# Autodesk Inventor assembly: Track Design 9-24-19
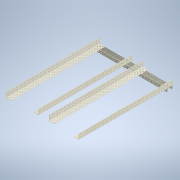
[picture p0: Inventor's stored thumbnail of the model, 180x180]
Saved by Autodesk Inventor 2020 (Build 240168000, 168)
## iProperties
Created: 2019-07-25
Part Number: Track Design 9-24-19
Document SubType Name: Assembly
Designer: Corey
Author: Corey
## Documents named in this file (3)
- C:\Users\Corey\Documents\Tower-Takeover-CAD\Parts\Dual Track.iam
- C:\Users\Corey\Documents\Tower-Takeover-CAD\Parts\Structure\90 Degree Brackets\Aluminum\Aluminum Angle 2x2x35.ipt
- C:\Users\Corey\Documents\Tower-Takeover-CAD\Parts\Structure\C-Channels\Aluminum\2-Wide\Aluminum C-Channel 1x2x1x27.ipt
## Components (5 placed, 2 different names)
1. Aluminum Angle 2x2x35:1 — Mate:6, Flush:11, Flush:12
2. Aluminum Angle 2x2x35:2 — Flush:17, Flush:18
3. Aluminum Angle 2x2x35:3 — Flush:15, Flush:16
4. Aluminum Angle 2x2x35:4
5. Aluminum C-Channel 1x2x1x27:1 — Mate:6, Flush:11, Flush:12, Flush:15, Flush:16, Flush:17, Flush:18
## Relationships (7: Flush 6, Mate 1)
- Mate:6: Aluminum Angle 2x2x35:1 ↔ Aluminum C-Channel 1x2x1x27:1
- Flush:11: Aluminum Angle 2x2x35:1 ↔ Aluminum C-Channel 1x2x1x27:1
- Flush:12: Aluminum Angle 2x2x35:1 ↔ Aluminum C-Channel 1x2x1x27:1
- Flush:15: Aluminum Angle 2x2x35:3 ↔ Aluminum C-Channel 1x2x1x27:1
- Flush:16: Aluminum Angle 2x2x35:3 ↔ Aluminum C-Channel 1x2x1x27:1
- Flush:17: Aluminum Angle 2x2x35:2 ↔ Aluminum C-Channel 1x2x1x27:1
- Flush:18: Aluminum Angle 2x2x35:2 ↔ Aluminum C-Channel 1x2x1x27:1
